# Autodesk Inventor assembly: calosc
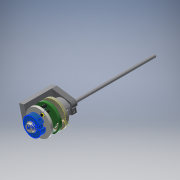
[picture p0: Inventor's stored thumbnail of the model, 180x180]
Saved by Autodesk Inventor 2017 (Build 210142000, 142)
## iProperties
Created: 2021-05-22
Part Number: calosc
Document SubType Name: Assembly
Designer: majch
Author: majch
## Documents named in this file (12)
- E:\inventor\mocowanie\calosc.iam
- E:\inventor\mocowanie\ogolny_walek-013.ipt
- E:\inventor\mocowanie\ogolny_walek.ipt
- E:\inventor\mocowanie\sprzeglo_03.ipt
- E:\inventor\mocowanie\sprzeglo_02.ipt
- E:\inventor\mocowanie\sprzeglo_01.ipt
- E:\inventor\mocowanie\waleczek_do_sprezyn_fi6.ipt
- E:\inventor\mocowanie\sprzeglo_04.ipt
- E:\inventor\mocowanie\walek popychajacy sprzeglo 01-02.ipt
- E:\inventor\mocowanie\baza.ipt
- E:\inventor\mocowanie\mocowanie walka.ipt
- E:\inventor\mocowanie\mocowanie uchwytu01.ipt
## Components (11 placed, 10 different names)
1. ogolny_walek-013:1 — Mate:2, Mate:3, Mate:8, Flush:6, Mate:12, Mate:16
2. sprzeglo_03:1 — Mate:3, Mate:6, Flush:3, Mate:9, Mate:10, Flush:6, Angle:2
3. sprzeglo_02:1 — Mate:2, Mate:5, Flush:4, Mate:10, Mate:18
4. waleczek_do_sprezyn_fi6:1 — Mate:6, Flush:3
5. waleczek_do_sprezyn_fi6:3 — Mate:5, Flush:4
6. sprzeglo_04:1 — Mate:8, Mate:9, Angle:2
7. baza:1 — Mate:13, Mate:14, Mate:15
8. mocowanie walka:1 — Mate:12, Mate:13, Mate:14, Mate:15, Angle:1
9. walek popychajacy sprzeglo 01-02:1 — Flush:7, Mate:17
10. sprzeglo_01:1 — Mate:16, Flush:7, Mate:17, Mate:18, Angle:1, Mate:19, Mate:20, Angle:3
11. mocowanie uchwytu01:1 — Mate:19, Mate:20, Angle:3
## Relationships (23: Mate 16, Flush 4, Angle 3)
- Mate:2: ogolny_walek-013:1 ↔ sprzeglo_02:1
- Mate:3: ogolny_walek-013:1 ↔ sprzeglo_03:1
- Mate:5: sprzeglo_02:1 ↔ waleczek_do_sprezyn_fi6:3
- Mate:6: sprzeglo_03:1 ↔ waleczek_do_sprezyn_fi6:1
- Flush:3: sprzeglo_03:1 ↔ waleczek_do_sprezyn_fi6:1
- Flush:4: sprzeglo_02:1 ↔ waleczek_do_sprezyn_fi6:3
- Mate:8: ogolny_walek-013:1 ↔ sprzeglo_04:1
- Mate:9: sprzeglo_03:1 ↔ sprzeglo_04:1
- Mate:10: sprzeglo_03:1 ↔ sprzeglo_02:1
- Flush:6: ogolny_walek-013:1 ↔ sprzeglo_03:1
- Mate:12: ogolny_walek-013:1 ↔ mocowanie walka:1
- Mate:13: baza:1 ↔ mocowanie walka:1
- Mate:14: baza:1 ↔ mocowanie walka:1
- Mate:15: baza:1 ↔ mocowanie walka:1
- Mate:16: ogolny_walek-013:1 ↔ sprzeglo_01:1
- Flush:7: walek popychajacy sprzeglo 01-02:1 ↔ sprzeglo_01:1
- Mate:17: walek popychajacy sprzeglo 01-02:1 ↔ sprzeglo_01:1
- Mate:18: sprzeglo_02:1 ↔ sprzeglo_01:1
- Angle:1 (30 deg): mocowanie walka:1 ↔ sprzeglo_01:1
- Angle:2 (-45 deg): sprzeglo_03:1 ↔ sprzeglo_04:1
- Mate:19: sprzeglo_01:1 ↔ mocowanie uchwytu01:1
- Mate:20: sprzeglo_01:1 ↔ mocowanie uchwytu01:1
- Angle:3 (0 deg): sprzeglo_01:1 ↔ mocowanie uchwytu01:1
